# Autodesk Inventor assembly: dc jack
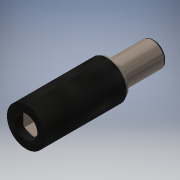
[picture p0: Inventor's stored thumbnail of the model, 180x180]
Saved by Autodesk Inventor 2019 (Build 230136000, 136)
## iProperties
Created: 2020-03-05
Part Number: dc jack
Document SubType Name: Assembly
Designer: ntb11189
Author: ntb11189
## Documents named in this file (3)
- N:\Sandpit\Callum Brooksby\Main Enclosure\Solar charger\dc jack.iam
- N:\Sandpit\Callum Brooksby\Main Enclosure\Solar charger\dc cover.ipt
- N:\Sandpit\Callum Brooksby\Main Enclosure\Solar charger\DC Power Plug 2.1x5.5mm Plug.ipt
## Components (2 placed, 2 different names)
1. dc cover:1 — Mate:1, Tangent:1
2. DC Power Plug 2.1x5.5mm Plug:1 — Mate:1, Tangent:1
## Relationships (2: Mate 1, Tangent 1)
- Mate:1: dc cover:1 ↔ DC Power Plug 2.1x5.5mm Plug:1
- Tangent:1 (-7 mm): dc cover:1 ↔ DC Power Plug 2.1x5.5mm Plug:1
